# Autodesk Inventor assembly: NDV-4000 Pipe flange 01
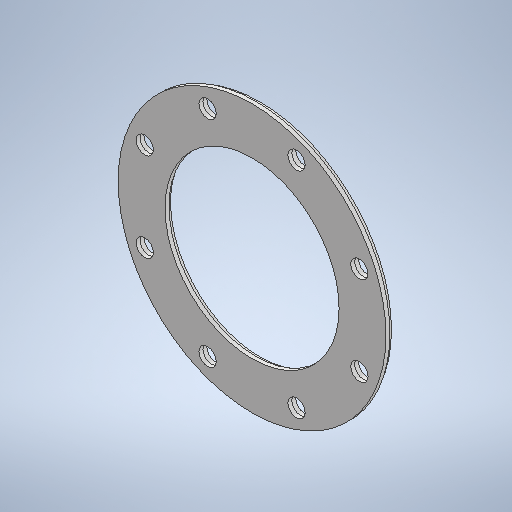
[picture p0: Inventor's stored thumbnail of the model, 512x512]
Saved by Autodesk Inventor 2026.2 (Build 302298000, 298)
## iProperties
Created: 2026-10-05
Part Number: NDV-4000 Pipe flange 01
Document SubType Name: Assembly
Designer: admin
Stock Number: Фланец трубы DN200
Author: admin
## Documents named in this file (3)
- C:\Users\admin\Documents\Inventor\NDV-DistribSystem\DRS_D1200\NDV-4000 Pipe flange 01.iam
- C:\Users\admin\Documents\Inventor\NDV-DistribSystem\DRS_D1200\NDV-4101 Pipe flange 01.ipt
- C:\Users\admin\Documents\Inventor\NDV-DistribSystem\DRS_D1200\NDV-4102 Pipe flange top 01.ipt
## Components (2 placed, 2 different names)
1. NDV-4101 Pipe flange 01:1 — Mate:1, Flush:1, Flush:2
2. NDV-4102 Pipe flange top 01:1 — Mate:1, Flush:1, Flush:2
## Relationships (3: Flush 2, Mate 1)
- Mate:1: NDV-4101 Pipe flange 01:1 ↔ NDV-4102 Pipe flange top 01:1
- Flush:1: NDV-4101 Pipe flange 01:1 ↔ NDV-4102 Pipe flange top 01:1
- Flush:2: NDV-4101 Pipe flange 01:1 ↔ NDV-4102 Pipe flange top 01:1
